# Autodesk Inventor assembly: voorwiel
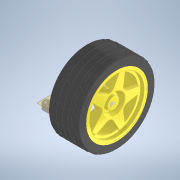
[picture p0: Inventor's stored thumbnail of the model, 180x180]
Saved by Autodesk Inventor 2022 (Build 260153000, 153)
## iProperties
Created: 2021-12-21
Part Number: voorwiel
Document SubType Name: Assembly
Designer: keemi
Author: keemi
## Documents named in this file (4)
- C:\Users\keemi\OneDrive\Bureaublad\repo's\projecten\Auto\modellen\inventor\auto moddel\voorwiel.iam
- C:\Users\keemi\OneDrive\Bureaublad\repo's\projecten\Auto\modellen\inventor\wheel-arduino-1.snapshot.2\Wheel ALL.ipt
- C:\Users\keemi\OneDrive\Bureaublad\repo's\projecten\Auto\modellen\inventor\auto moddel\wielas.ipt
- C:\Users\keemi\OneDrive\Bureaublad\repo's\projecten\Auto\modellen\inventor\auto moddel\STUURAS.ipt
## Components (3 placed, 3 different names)
1. Wheel ALL:1 — Mate:1, Mate:4
2. wielas:1 — Mate:2, Mate:3, Mate:4
3. STUURAS:1 — Mate:1, Mate:2, Mate:3
## Relationships (4: Mate 4)
- Mate:1: Wheel ALL:1 ↔ STUURAS:1
- Mate:2: wielas:1 ↔ STUURAS:1
- Mate:3: wielas:1 ↔ STUURAS:1
- Mate:4: Wheel ALL:1 ↔ wielas:1
